# Autodesk Inventor assembly: All Keys
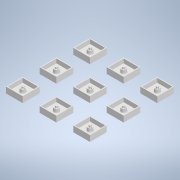
[picture p0: Inventor's stored thumbnail of the model, 180x180]
Saved by Autodesk Inventor 2021.1 (Build 251245000, 245)
## iProperties
Created: 2020-08-05
Part Number: All Keys
Document SubType Name: Assembly
Designer: adick
Author: adick
## Documents named in this file (2)
- C:\Users\adick\Documents\Kerbal Kontroller\Design\Final\3d Print\All Keys.iam
- C:\Users\adick\Documents\Kerbal Kontroller\Design\Final\3d Print\test2.ipt
## Components (9 placed, 1 different names)
1. test2:1
2. test2:2
3. test2:3
4. test2:4
5. test2:5
6. test2:6
7. test2:7
8. test2:8
9. test2:9
## Component patterns: (3 elements), (3 elements, first: test2:1), Component Pattern 1:2 (3 elements), Component Pattern 1:3 (3 elements)
